# Autodesk Inventor assembly: PotentiometerAssembly
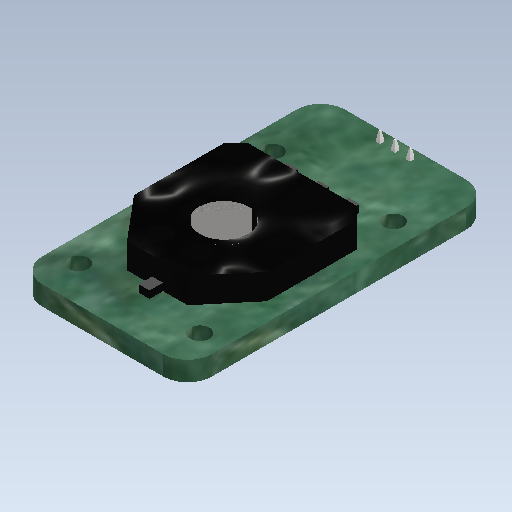
[picture p0: Inventor's stored thumbnail of the model, 512x512]
Saved by Autodesk Inventor 2020 (Build 240168000, 168)
## iProperties
Created: 2020-01-18
Part Number: PotentiometerAssembly
Document SubType Name: Assembly
Designer: sami_
Author: sami_
## Documents named in this file (5)
- C:\Users\ttail\Downloads\Inventor Hand\Curved Hand V1.4\Workgroups\NotInProject\INDEX\PotentiometerAssembly.iam
- C:\Users\ttail\Downloads\Inventor Hand\Curved Hand V1.4\Workgroups\NotInProject\INDEX\potentiometerbody.ipt
- C:\Users\ttail\Downloads\Inventor Hand\Curved Hand V1.4\Workgroups\NotInProject\INDEX\potentiometerspinny.ipt
- C:\Users\ttail\Downloads\Inventor Hand\Curved Hand V1.4\Workgroups\NotInProject\INDEX\potentiometerpcb.ipt
- C:\Users\ttail\Downloads\Inventor Hand\Curved Hand V1.4\Workgroups\NotInProject\530470310.ipt
## Components (4 placed, 4 different names)
1. potentiometerbody:1 — Rotational:1, Rigid:1
2. potentiometerspinny:1 — Rotational:1
3. potentiometerpcb:1 — Rigid:1, Rigid:2
4. 530470310:3 — Rigid:2
## Relationships (3: WeldJoint 2, RevoluteJoint 1)
- Rotational:1 [RevoluteJoint] (0.02 mm): potentiometerbody:1 ↔ potentiometerspinny:1
- Rigid:1 [WeldJoint]: potentiometerbody:1 ↔ potentiometerpcb:1
- Rigid:2 [WeldJoint]: potentiometerpcb:1 ↔ 530470310:3
